# Autodesk Inventor assembly: ball_transfer
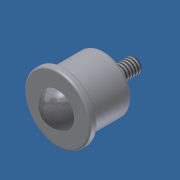
[picture p0: Inventor's stored thumbnail of the model, 180x180]
Saved by Autodesk Inventor 2011 (Build 150239000, 239)
## iProperties
Created: 2011-01-09
Part Number: ball_transfer
Document SubType Name: Assembly
Designer: Antonella Wilby
Author: Antonella Wilby
## Documents named in this file (3)
- C:\Documents and Settings\Antonella Wilby\My Documents\Inventor\GCC_Robotics_IGVC_2011\Ball Caster\ball_transfer.iam
- C:\Documents and Settings\Antonella Wilby\My Documents\Inventor\GCC_Robotics_IGVC_2011\Ball Caster\ball_bearing.ipt
- C:\Documents and Settings\Antonella Wilby\My Documents\Inventor\GCC_Robotics_IGVC_2011\Ball Caster\transfer_housing.ipt
## Components (2 placed, 2 different names)
1. ball_bearing:1 — Mate:1
2. transfer_housing:1 — Mate:1
## Relationships (1: Mate 1)
- Mate:1: ball_bearing:1 ↔ transfer_housing:1
